# Autodesk Inventor assembly: Gestikulaser
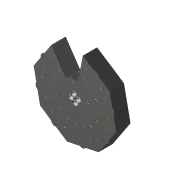
[picture p0: Inventor's stored thumbnail of the model, 180x180]
Saved by Autodesk Inventor 2018 (Build 220112000, 112)
## iProperties
Created: 2018-11-01
Part Number: Gestikulaser
Material: Generisch
Document SubType Name: Assembly
Designer: M.Knabel
Author: M.Knabel
## Documents named in this file (3)
- C:\Users\knabe\Documents\GitHub\COSIMA-Laserstar\CAD\Gestikulaser.iam
- C:\Users\knabe\Documents\GitHub\COSIMA-Laserstar\CAD\Oktokommander\Oktokommander.iam
- C:\Users\knabe\Documents\GitHub\COSIMA-Laserstar\CAD\Detektormodul\Detektormodul.iam
## Components (8 placed, 2 different names)
1. Oktokommander:1 [sub-assembly] — Fluchtend:1, Passend:1, Fluchtend:3, Fluchtend:14, Passend:6, Passend:7, Passend:8, Passend:9, Fluchtend:4, Passend:10, Fluchtend:5, Passend:11, Fluchtend:6, Fluchtend:7, Passend:12, Passend:13, Fluchtend:8, Fluchtend:9, Fluchtend:12, Passend:14
2. Detektormodul:2 [sub-assembly] — Passend:1, Fluchtend:2, Fluchtend:14
3. Detektormodul:3 [sub-assembly] — Fluchtend:2, Fluchtend:3, Passend:9, Fluchtend:4
4. Detektormodul:5 [sub-assembly] — Passend:13, Fluchtend:9, Fluchtend:10
5. Detektormodul:6 [sub-assembly] — Passend:12, Fluchtend:8, Fluchtend:10, Fluchtend:11
6. Detektormodul:7 [sub-assembly] — Passend:11, Fluchtend:6, Fluchtend:7, Fluchtend:11, Fluchtend:13
7. Detektormodul:8 [sub-assembly] — Fluchtend:1, Passend:10, Fluchtend:5
8. Detektormodul:9 [sub-assembly] — Fluchtend:12, Passend:14, Fluchtend:13
## Relationships (24: Flush 14, Mate 10)
- Fluchtend:1 [Flush]: Oktokommander:1 ↔ Detektormodul:8
- Passend:1 [Mate]: Oktokommander:1 ↔ Detektormodul:2
- Fluchtend:2 [Flush]: Detektormodul:2 ↔ Detektormodul:3
- Fluchtend:3 [Flush]: Oktokommander:1 ↔ Detektormodul:3
- Fluchtend:14 [Flush]: Oktokommander:1 ↔ Detektormodul:2
- Passend:6 [Mate]: Oktokommander:1
- Passend:7 [Mate]: Oktokommander:1
- Passend:8 [Mate]: Oktokommander:1
- Passend:9 [Mate]: Oktokommander:1 ↔ Detektormodul:3
- Fluchtend:4 [Flush]: Oktokommander:1 ↔ Detektormodul:3
- Passend:10 [Mate]: Oktokommander:1 ↔ Detektormodul:8
- Fluchtend:5 [Flush]: Oktokommander:1 ↔ Detektormodul:8
- Passend:11 [Mate]: Oktokommander:1 ↔ Detektormodul:7
- Fluchtend:6 [Flush]: Oktokommander:1 ↔ Detektormodul:7
- Fluchtend:7 [Flush]: Oktokommander:1 ↔ Detektormodul:7
- Passend:12 [Mate]: Oktokommander:1 ↔ Detektormodul:6
- Passend:13 [Mate]: Oktokommander:1 ↔ Detektormodul:5
- Fluchtend:8 [Flush]: Oktokommander:1 ↔ Detektormodul:6
- Fluchtend:9 [Flush]: Oktokommander:1 ↔ Detektormodul:5
- Fluchtend:10 [Flush]: Detektormodul:5 ↔ Detektormodul:6
- Fluchtend:11 [Flush]: Detektormodul:6 ↔ Detektormodul:7
- Fluchtend:12 [Flush]: Oktokommander:1 ↔ Detektormodul:9
- Passend:14 [Mate]: Oktokommander:1 ↔ Detektormodul:9
- Fluchtend:13 [Flush]: Detektormodul:7 ↔ Detektormodul:9
